# Autodesk Inventor assembly: 胴体_1
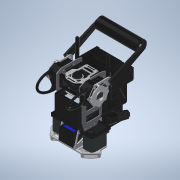
[picture p0: Inventor's stored thumbnail of the model, 180x180]
Saved by Autodesk Inventor 2020 (Build 240168000, 168)
## iProperties
Created: 2016-05-03
Part Number: 胴体_1
Document SubType Name: Assembly
Designer: hiroaki
Mass: 1394.39 g
Surface Area: 4542.63 cm^2
Volume: 847.153 cm^3
Density: 1.64598 g/cm^3
Author: hiroaki
## Documents named in this file (26)
- C:\Users\Masato\Documents\Inventor\CIT Brains_Inventor\OpenPlatform_ver3_0\上半身\胴体\胴体_1.iam
- C:\Users\Masato\Documents\Inventor\CIT Brains_Inventor\OpenPlatform_ver3_0\既製品\B3M11xx.ipt
- C:\Users\Masato\Documents\Inventor\CIT Brains_Inventor\OpenPlatform_ver3_0\既製品\B3M10xx.ipt
- C:\Users\Masato\Documents\Inventor\CIT Brains_Inventor\OpenPlatform_ver3_0\上半身\胴体\胴体_メインフレーム_1_1.ipt
- C:\Users\Masato\Documents\Inventor\CIT Brains_Inventor\OpenPlatform_ver3_0\下半身\付け根ロール\付け根ロール_サブフレーム_1_3.ipt
- C:\Users\Masato\Documents\Inventor\CIT Brains_Inventor\OpenPlatform_ver3_0\上半身\胴体\胴体_メインフレーム_1_2.ipt
- C:\Users\Masato\Documents\Inventor\CIT Brains_Inventor\OpenPlatform_ver3_0\上半身\胴体\胴体_サブフレーム_1_1.ipt
- C:\Users\Masato\Documents\Inventor\CIT Brains_Inventor\OpenPlatform_ver3_0\上半身\胴体\胴体_サブフレーム_1_2.ipt
- C:\Users\Masato\Documents\Inventor\CIT Brains_Inventor\OpenPlatform_ver3_0\上半身\胴体\胴体_サブフレーム_1_3.ipt
- C:\Users\Masato\Documents\Inventor\CIT Brains_Inventor\OpenPlatform_ver3_0\上半身\胴体\胴体_サブフレーム_1_4.ipt
- C:\Users\Masato\Documents\Inventor\CIT Brains_Inventor\OpenPlatform_ver3_0\上半身\胴体\胴体_サブフレーム_1_1_MIR.ipt
- C:\Users\Masato\Documents\Inventor\CIT Brains_Inventor\OpenPlatform_ver3_0\上半身\胴体\胴体_サブフレーム_1_9.ipt
- C:\Users\Masato\Documents\Inventor\CIT Brains_Inventor\OpenPlatform_ver3_0\上半身\胴体\胴体_メインフレーム_1_12.ipt
- C:\Users\Masato\Documents\Inventor\CIT Brains_Inventor\OpenPlatform_ver3_0\上半身\胴体\胴体_メインフレーム_1_13.ipt
- C:\Users\Masato\Documents\Inventor\CIT Brains_Inventor\OpenPlatform_ver3_0\上半身\胴体\胴体_サブフレーム_1_10.ipt
- C:\Users\Masato\Documents\Inventor\CIT Brains_Inventor\OpenPlatform_ver3_0\既製品\MSU-306-03.ipt
- C:\Users\Masato\Documents\Inventor\CIT Brains_Inventor\OpenPlatform_ver3_0\既製品\ALSFB6-66.ipt
- C:\Users\Masato\Documents\Inventor\CIT Brains_Inventor\OpenPlatform_ver3_0\上半身\胴体\胴体_サブフレーム_1_12.ipt
- C:\Users\Masato\Documents\Inventor\CIT Brains_Inventor\OpenPlatform_ver3_0\上半身\胴体\胴体_サブフレーム_1_4_MIR.ipt
- C:\Users\Masato\Documents\Inventor\CIT Brains_Inventor\OpenPlatform_ver3_0\上半身\胴体\RearBumper_Lower.ipt
- C:\Users\Masato\Documents\Inventor\CIT Brains_Inventor\OpenPlatform_ver3_0\上半身\胴体\RearBumper_Lower_MIR.ipt
- C:\Users\Masato\Documents\Inventor\CIT Brains_Inventor\OpenPlatform_ver3_0\上半身\胴体\FrontBumper_MIR.iam
- C:\Users\Masato\Documents\Inventor\CIT Brains_Inventor\OpenPlatform_ver3_0\上半身\胴体\FrontBumper.iam
- C:\Users\Masato\Documents\Inventor\CIT Brains_Inventor\OpenPlatform_ver3_0\既製品\SGB-100.ipt
- C:\Users\Masato\Documents\Inventor\CIT Brains_Inventor\OpenPlatform_ver3_0\上半身\Cockpit\Cockpit.iam
- C:\Users\Masato\Documents\Inventor\CIT Brains_Inventor\OpenPlatform_ver3_0\既製品\AETTF8-130-M3-N3.ipt
## Components (61 placed, 24 different names)
1. 胴体_メインフレーム_1_1:1 — 挿入:1, 挿入:2, 挿入:3, 挿入:4, 挿入:5, 挿入:6, 挿入:43, 挿入:44, 挿入:120, 挿入:121, 挿入:194, 挿入:195, 挿入:196, 挿入:197, 挿入:198, 挿入:199, 挿入:200, 挿入:201, メイト:18
2. 付け根ロール_サブフレーム_1_3:1 — 挿入:218, 挿入:219, 挿入:220, 挿入:221
3. 胴体_メインフレーム_1_2:1 — 挿入:23, 挿入:24, 挿入:25, 挿入:28
4. 胴体_メインフレーム_1_12:1 — 挿入:148, 挿入:149, 挿入:150, 挿入:151, メイト:13, メイト:16
5. 胴体_サブフレーム_1_1:1 — 挿入:43, 挿入:44, メイト:10, メイト:11, 挿入:275, 挿入:276
6. 胴体_サブフレーム_1_2:1 — フラッシュ:1, メイト:3, メイト:4
7. 胴体_サブフレーム_1_3:1 — 挿入:150, 挿入:151, 挿入:162, 挿入:163, 挿入:168, 挿入:169, 挿入:192, 挿入:193, 挿入:228, 挿入:229, メイト:4, 挿入:236, メイト:12, フラッシュ:2
8. 胴体_サブフレーム_1_4:1 — 挿入:57, 挿入:58, 挿入:148, 挿入:149, 挿入:152, 挿入:153, 挿入:206, 挿入:207, 挿入:208, 挿入:209, 挿入:248, 挿入:249, 角度:47, 角度:48
9. 胴体_サブフレーム_1_9:1 — 挿入:133, 挿入:134, 挿入:135
10. 胴体_サブフレーム_1_10:1 — 挿入:173, 挿入:174, 挿入:175, 挿入:176, 挿入:179, 挿入:188, 挿入:189
11. 胴体_サブフレーム_1_12:1 — 挿入:250, 挿入:251
12. 胴体_メインフレーム_1_13:1 — 挿入:188, 挿入:189, 挿入:190, 挿入:191, 挿入:192, 挿入:193, 挿入:277
13. B3M11xx:5 — 挿入:175, 挿入:176, 挿入:179
14. B3M11xx:4 — 挿入:57, 挿入:58, 挿入:133, 挿入:134, 挿入:135, 角度:31, 角度:39
15. B3M11xx:3 — 角度:1, 挿入:130, 挿入:131, 挿入:132, 挿入:264, 挿入:265, 挿入:266
16. B3M11xx:2 — 挿入:2, 挿入:4, 挿入:5, 挿入:23, 挿入:25, 角度:23, 角度:43
17. B3M11xx:1 — 角度:1, 挿入:1, 挿入:3, 挿入:6, 挿入:24, 挿入:28
18. MSU-306-03:1 — 挿入:200, 挿入:218, 角度:27, 角度:29
19. MSU-306-03:2 — 挿入:196, 挿入:222, 角度:25, 角度:28, 角度:43
20. MSU-306-03:3 — 挿入:198, 挿入:220, 角度:29
21. MSU-306-03:4 — 挿入:199, 挿入:219, 角度:30
22. MSU-306-03:5 — 挿入:217, 角度:34, 挿入:272
23. MSU-306-03:6 — 挿入:216, 角度:42, 挿入:271
24. MSU-306-03:7 — 挿入:197, 挿入:225, 角度:26
25. MSU-306-03:8 — 挿入:201, 挿入:221, 角度:28, 角度:30
26. MSU-306-03:9 — 挿入:206, 挿入:212, 角度:40
27. MSU-306-03:10 — 挿入:215, 角度:41, 挿入:269
28. MSU-306-03:11 — 挿入:214, 角度:33, 角度:34, 挿入:270
29. MSU-306-03:12 — 挿入:195, 挿入:224, 角度:25
30. MSU-306-03:13 — 挿入:207, 挿入:213, 角度:32
31. MSU-306-03:14 — 挿入:208, 挿入:211, 角度:31, 角度:32, 角度:33
32. MSU-306-03:15 — 挿入:209, 挿入:210, 角度:39, 角度:40, 角度:41, 角度:42
33. MSU-306-03:16 — 挿入:194, 挿入:223, 角度:23, 角度:26, 角度:27
34. ALSFB6-66:1 — 挿入:229, 挿入:230, メイト:3
35. ALSFB6-66:2 — 挿入:227, 挿入:228, メイト:1, メイト:2
36. ALSFB6-66:3 — メイト:10, メイト:11, 挿入:235, 挿入:236
37. MSU-306-03:17 — 挿入:252, 挿入:262
38. MSU-306-03:18 — 挿入:249, 挿入:251, 角度:48
39. MSU-306-03:19 — 挿入:253, 挿入:263
40. MSU-306-03:20 — 挿入:248, 挿入:250, 角度:47
41. 胴体_サブフレーム_1_12:2 — 挿入:252, 挿入:253, 挿入:279, 挿入:280
42. 胴体_メインフレーム_1_13:2 — 挿入:168, 挿入:169, 挿入:170, 挿入:171, 挿入:173, 挿入:174, 挿入:278
43. 胴体_メインフレーム_1_12:2 — 挿入:152, 挿入:153, 挿入:162, 挿入:163
44. 胴体_メインフレーム_1_12:3 — 挿入:156, 挿入:157, 挿入:267, 挿入:268
45. 胴体_メインフレーム_1_12:4 — 挿入:160, 挿入:161, 挿入:260, 挿入:261, メイト:15, メイト:17
46. 胴体_サブフレーム_1_9:2 — 挿入:130, 挿入:131, 挿入:132
47. 付け根ロール_サブフレーム_1_3:2 — 挿入:222, 挿入:223, 挿入:224, 挿入:225
48. 付け根ロール_サブフレーム_1_3:3 — 挿入:210, 挿入:211, 挿入:212, 挿入:213
49. 付け根ロール_サブフレーム_1_3:4 — 挿入:214, 挿入:215, 挿入:216, 挿入:217
50. 胴体_サブフレーム_1_1_MIR:1 — 挿入:120, 挿入:121, メイト:7, 挿入:273, 挿入:274
51. 胴体_サブフレーム_1_2:2 — メイト:1, フラッシュ:1, メイト:2, メイト:5, メイト:7
52. 胴体_サブフレーム_1_3:2 — 挿入:156, 挿入:157, 挿入:160, 挿入:161, 挿入:170, 挿入:171, 挿入:190, 挿入:191, 挿入:227, 挿入:230, メイト:5, 挿入:235, メイト:14, メイト:19
53. 胴体_サブフレーム_1_4_MIR:1 — 挿入:260, 挿入:261, 挿入:262, 挿入:263, 挿入:264, 挿入:265, 挿入:266, 挿入:267, 挿入:268, 挿入:269, 挿入:270, 挿入:271, 挿入:272
54. RearBumper_Lower:1 — 挿入:275, 挿入:276
55. RearBumper_Lower_MIR:1 — 挿入:273, 挿入:274
56. FrontBumper_MIR:1 [sub-assembly] — メイト:12, メイト:13, メイト:16
57. FrontBumper:1 [sub-assembly] — メイト:14, メイト:15, メイト:17
58. 胴体_サブフレーム_1_10:2 — 挿入:277, 挿入:278
59. SGB-100:1 — 挿入:280
60. Cockpit:1 [sub-assembly] — フラッシュ:2, メイト:18, メイト:19
61. AETTF8-130-M3-N3:1 — 挿入:279
## Relationships (147: Insert 110, Angle 19, Mate 16, Flush 2)
- 角度:1 [Angle] (0 deg): B3M11xx:3 ↔ B3M11xx:1
- 挿入:1 [Insert]: 胴体_メインフレーム_1_1:1 ↔ B3M11xx:1
- 挿入:2 [Insert]: 胴体_メインフレーム_1_1:1 ↔ B3M11xx:2
- 挿入:3 [Insert]: 胴体_メインフレーム_1_1:1 ↔ B3M11xx:1
- 挿入:4 [Insert]: 胴体_メインフレーム_1_1:1 ↔ B3M11xx:2
- 挿入:5 [Insert]: 胴体_メインフレーム_1_1:1 ↔ B3M11xx:2
- 挿入:6 [Insert]: 胴体_メインフレーム_1_1:1 ↔ B3M11xx:1
- 挿入:23 [Insert]: 胴体_メインフレーム_1_2:1 ↔ B3M11xx:2
- 挿入:24 [Insert]: 胴体_メインフレーム_1_2:1 ↔ B3M11xx:1
- 挿入:25 [Insert]: 胴体_メインフレーム_1_2:1 ↔ B3M11xx:2
- 挿入:28 [Insert]: 胴体_メインフレーム_1_2:1 ↔ B3M11xx:1
- 挿入:43 [Insert]: 胴体_メインフレーム_1_1:1 ↔ 胴体_サブフレーム_1_1:1
- 挿入:44 [Insert]: 胴体_メインフレーム_1_1:1 ↔ 胴体_サブフレーム_1_1:1
- 挿入:57 [Insert]: 胴体_サブフレーム_1_4:1 ↔ B3M11xx:4
- 挿入:58 [Insert]: 胴体_サブフレーム_1_4:1 ↔ B3M11xx:4
- 挿入:120 [Insert]: 胴体_メインフレーム_1_1:1 ↔ 胴体_サブフレーム_1_1_MIR:1
- 挿入:121 [Insert]: 胴体_メインフレーム_1_1:1 ↔ 胴体_サブフレーム_1_1_MIR:1
- 挿入:130 [Insert]: B3M11xx:3 ↔ 胴体_サブフレーム_1_9:2
- 挿入:131 [Insert]: B3M11xx:3 ↔ 胴体_サブフレーム_1_9:2
- 挿入:132 [Insert]: B3M11xx:3 ↔ 胴体_サブフレーム_1_9:2
- 挿入:133 [Insert]: 胴体_サブフレーム_1_9:1 ↔ B3M11xx:4
- 挿入:134 [Insert]: 胴体_サブフレーム_1_9:1 ↔ B3M11xx:4
- 挿入:135 [Insert]: 胴体_サブフレーム_1_9:1 ↔ B3M11xx:4
- 挿入:148 [Insert]: 胴体_メインフレーム_1_12:1 ↔ 胴体_サブフレーム_1_4:1
- 挿入:149 [Insert]: 胴体_メインフレーム_1_12:1 ↔ 胴体_サブフレーム_1_4:1
- 挿入:150 [Insert]: 胴体_メインフレーム_1_12:1 ↔ 胴体_サブフレーム_1_3:1
- 挿入:151 [Insert]: 胴体_メインフレーム_1_12:1 ↔ 胴体_サブフレーム_1_3:1
- 挿入:152 [Insert]: 胴体_サブフレーム_1_4:1 ↔ 胴体_メインフレーム_1_12:2
- 挿入:153 [Insert]: 胴体_サブフレーム_1_4:1 ↔ 胴体_メインフレーム_1_12:2
- 挿入:156 [Insert]: 胴体_メインフレーム_1_12:3 ↔ 胴体_サブフレーム_1_3:2
- 挿入:157 [Insert]: 胴体_メインフレーム_1_12:3 ↔ 胴体_サブフレーム_1_3:2
- 挿入:160 [Insert]: 胴体_メインフレーム_1_12:4 ↔ 胴体_サブフレーム_1_3:2
- 挿入:161 [Insert]: 胴体_メインフレーム_1_12:4 ↔ 胴体_サブフレーム_1_3:2
- 挿入:162 [Insert]: 胴体_サブフレーム_1_3:1 ↔ 胴体_メインフレーム_1_12:2
- 挿入:163 [Insert]: 胴体_サブフレーム_1_3:1 ↔ 胴体_メインフレーム_1_12:2
- 挿入:168 [Insert]: 胴体_サブフレーム_1_3:1 ↔ 胴体_メインフレーム_1_13:2
- 挿入:169 [Insert]: 胴体_サブフレーム_1_3:1 ↔ 胴体_メインフレーム_1_13:2
- 挿入:170 [Insert]: 胴体_メインフレーム_1_13:2 ↔ 胴体_サブフレーム_1_3:2
- 挿入:171 [Insert]: 胴体_メインフレーム_1_13:2 ↔ 胴体_サブフレーム_1_3:2
- 挿入:173 [Insert]: 胴体_サブフレーム_1_10:1 ↔ 胴体_メインフレーム_1_13:2
- 挿入:174 [Insert]: 胴体_サブフレーム_1_10:1 ↔ 胴体_メインフレーム_1_13:2
- 挿入:175 [Insert]: 胴体_サブフレーム_1_10:1 ↔ B3M11xx:5
- 挿入:176 [Insert]: 胴体_サブフレーム_1_10:1 ↔ B3M11xx:5
- 挿入:179 [Insert]: 胴体_サブフレーム_1_10:1 ↔ B3M11xx:5
- 挿入:188 [Insert]: 胴体_サブフレーム_1_10:1 ↔ 胴体_メインフレーム_1_13:1
- 挿入:189 [Insert]: 胴体_サブフレーム_1_10:1 ↔ 胴体_メインフレーム_1_13:1
- 挿入:190 [Insert]: 胴体_メインフレーム_1_13:1 ↔ 胴体_サブフレーム_1_3:2
- 挿入:191 [Insert]: 胴体_メインフレーム_1_13:1 ↔ 胴体_サブフレーム_1_3:2
- 挿入:192 [Insert]: 胴体_サブフレーム_1_3:1 ↔ 胴体_メインフレーム_1_13:1
- 挿入:193 [Insert]: 胴体_サブフレーム_1_3:1 ↔ 胴体_メインフレーム_1_13:1
- 挿入:194 [Insert]: 胴体_メインフレーム_1_1:1 ↔ MSU-306-03:16
- 挿入:195 [Insert]: 胴体_メインフレーム_1_1:1 ↔ MSU-306-03:12
- 挿入:196 [Insert]: 胴体_メインフレーム_1_1:1 ↔ MSU-306-03:2
- 挿入:197 [Insert]: 胴体_メインフレーム_1_1:1 ↔ MSU-306-03:7
- 挿入:198 [Insert]: 胴体_メインフレーム_1_1:1 ↔ MSU-306-03:3
- 挿入:199 [Insert]: 胴体_メインフレーム_1_1:1 ↔ MSU-306-03:4
- 挿入:200 [Insert]: 胴体_メインフレーム_1_1:1 ↔ MSU-306-03:1
- 挿入:201 [Insert]: 胴体_メインフレーム_1_1:1 ↔ MSU-306-03:8
- 挿入:206 [Insert]: 胴体_サブフレーム_1_4:1 ↔ MSU-306-03:9
- 挿入:207 [Insert]: 胴体_サブフレーム_1_4:1 ↔ MSU-306-03:13
- 挿入:208 [Insert]: 胴体_サブフレーム_1_4:1 ↔ MSU-306-03:14
- 挿入:209 [Insert]: 胴体_サブフレーム_1_4:1 ↔ MSU-306-03:15
- 挿入:210 [Insert]: MSU-306-03:15 ↔ 付け根ロール_サブフレーム_1_3:3
- 挿入:211 [Insert]: MSU-306-03:14 ↔ 付け根ロール_サブフレーム_1_3:3
- 挿入:212 [Insert]: MSU-306-03:9 ↔ 付け根ロール_サブフレーム_1_3:3
- 挿入:213 [Insert]: MSU-306-03:13 ↔ 付け根ロール_サブフレーム_1_3:3
- 挿入:214 [Insert]: MSU-306-03:11 ↔ 付け根ロール_サブフレーム_1_3:4
- 挿入:215 [Insert]: MSU-306-03:10 ↔ 付け根ロール_サブフレーム_1_3:4
- 挿入:216 [Insert]: MSU-306-03:6 ↔ 付け根ロール_サブフレーム_1_3:4
- 挿入:217 [Insert]: MSU-306-03:5 ↔ 付け根ロール_サブフレーム_1_3:4
- 挿入:218 [Insert]: 付け根ロール_サブフレーム_1_3:1 ↔ MSU-306-03:1
- 挿入:219 [Insert]: 付け根ロール_サブフレーム_1_3:1 ↔ MSU-306-03:4
- 挿入:220 [Insert]: 付け根ロール_サブフレーム_1_3:1 ↔ MSU-306-03:3
- 挿入:221 [Insert]: 付け根ロール_サブフレーム_1_3:1 ↔ MSU-306-03:8
- 挿入:222 [Insert]: MSU-306-03:2 ↔ 付け根ロール_サブフレーム_1_3:2
- 挿入:223 [Insert]: MSU-306-03:16 ↔ 付け根ロール_サブフレーム_1_3:2
- 挿入:224 [Insert]: MSU-306-03:12 ↔ 付け根ロール_サブフレーム_1_3:2
- 挿入:225 [Insert]: MSU-306-03:7 ↔ 付け根ロール_サブフレーム_1_3:2
- 角度:23 [Angle] (0 deg): B3M11xx:2 ↔ MSU-306-03:16
- 角度:25 [Angle] (0 deg): MSU-306-03:2 ↔ MSU-306-03:12
- 角度:26 [Angle] (0 deg): MSU-306-03:7 ↔ MSU-306-03:16
- 角度:27 [Angle] (0 deg): MSU-306-03:1 ↔ MSU-306-03:16
- 角度:28 [Angle] (0 deg): MSU-306-03:2 ↔ MSU-306-03:8
- 角度:29 [Angle] (0 deg): MSU-306-03:1 ↔ MSU-306-03:3
- 角度:30 [Angle] (0 deg): MSU-306-03:4 ↔ MSU-306-03:8
- 角度:31 [Angle] (0 deg): B3M11xx:4 ↔ MSU-306-03:14
- 角度:32 [Angle] (0 deg): MSU-306-03:13 ↔ MSU-306-03:14
- 角度:33 [Angle] (0 deg): MSU-306-03:11 ↔ MSU-306-03:14
- 角度:34 [Angle] (0 deg): MSU-306-03:5 ↔ MSU-306-03:11
- 挿入:227 [Insert]: ALSFB6-66:2 ↔ 胴体_サブフレーム_1_3:2
- 挿入:228 [Insert]: 胴体_サブフレーム_1_3:1 ↔ ALSFB6-66:2
- 挿入:229 [Insert]: 胴体_サブフレーム_1_3:1 ↔ ALSFB6-66:1
- 挿入:230 [Insert]: ALSFB6-66:1 ↔ 胴体_サブフレーム_1_3:2
- メイト:1 [Mate] (0.005 mm): ALSFB6-66:2 ↔ 胴体_サブフレーム_1_2:2
- フラッシュ:1 [Flush]: 胴体_サブフレーム_1_2:1 ↔ 胴体_サブフレーム_1_2:2
- メイト:2 [Mate] (0.05 mm): ALSFB6-66:2 ↔ 胴体_サブフレーム_1_2:2
- メイト:3 [Mate] (0.005 mm): 胴体_サブフレーム_1_2:1 ↔ ALSFB6-66:1
- メイト:4 [Mate]: 胴体_サブフレーム_1_2:1 ↔ 胴体_サブフレーム_1_3:1
- メイト:5 [Mate]: 胴体_サブフレーム_1_2:2 ↔ 胴体_サブフレーム_1_3:2
- メイト:7 [Mate]: 胴体_サブフレーム_1_1_MIR:1 ↔ 胴体_サブフレーム_1_2:2
- メイト:10 [Mate] (0.005 mm): 胴体_サブフレーム_1_1:1 ↔ ALSFB6-66:3
- メイト:11 [Mate] (0.005 mm): 胴体_サブフレーム_1_1:1 ↔ ALSFB6-66:3
- 挿入:235 [Insert]: ALSFB6-66:3 ↔ 胴体_サブフレーム_1_3:2
- 挿入:236 [Insert]: 胴体_サブフレーム_1_3:1 ↔ ALSFB6-66:3
- 挿入:248 [Insert]: 胴体_サブフレーム_1_4:1 ↔ MSU-306-03:20
- 挿入:249 [Insert]: 胴体_サブフレーム_1_4:1 ↔ MSU-306-03:18
- 挿入:250 [Insert]: 胴体_サブフレーム_1_12:1 ↔ MSU-306-03:20
- 挿入:251 [Insert]: 胴体_サブフレーム_1_12:1 ↔ MSU-306-03:18
- 挿入:252 [Insert]: MSU-306-03:17 ↔ 胴体_サブフレーム_1_12:2
- 挿入:253 [Insert]: MSU-306-03:19 ↔ 胴体_サブフレーム_1_12:2
- 角度:39 [Angle] (0 deg): B3M11xx:4 ↔ MSU-306-03:15
- 角度:40 [Angle] (0 deg): MSU-306-03:9 ↔ MSU-306-03:15
- 角度:41 [Angle] (0 deg): MSU-306-03:10 ↔ MSU-306-03:15
- 角度:42 [Angle] (0 deg): MSU-306-03:6 ↔ MSU-306-03:15
- 角度:43 [Angle] (0 deg): B3M11xx:2 ↔ MSU-306-03:2
- 角度:47 [Angle] (0 deg): 胴体_サブフレーム_1_4:1 ↔ MSU-306-03:20
- 角度:48 [Angle] (0 deg): 胴体_サブフレーム_1_4:1 ↔ MSU-306-03:18
- 挿入:260 [Insert]: 胴体_メインフレーム_1_12:4 ↔ 胴体_サブフレーム_1_4_MIR:1
- 挿入:261 [Insert]: 胴体_メインフレーム_1_12:4 ↔ 胴体_サブフレーム_1_4_MIR:1
- 挿入:262 [Insert]: MSU-306-03:17 ↔ 胴体_サブフレーム_1_4_MIR:1
- 挿入:263 [Insert]: MSU-306-03:19 ↔ 胴体_サブフレーム_1_4_MIR:1
- 挿入:264 [Insert]: B3M11xx:3 ↔ 胴体_サブフレーム_1_4_MIR:1
- 挿入:265 [Insert]: B3M11xx:3 ↔ 胴体_サブフレーム_1_4_MIR:1
- 挿入:266 [Insert]: B3M11xx:3 ↔ 胴体_サブフレーム_1_4_MIR:1
- 挿入:267 [Insert]: 胴体_メインフレーム_1_12:3 ↔ 胴体_サブフレーム_1_4_MIR:1
- 挿入:268 [Insert]: 胴体_メインフレーム_1_12:3 ↔ 胴体_サブフレーム_1_4_MIR:1
- 挿入:269 [Insert]: MSU-306-03:10 ↔ 胴体_サブフレーム_1_4_MIR:1
- 挿入:270 [Insert]: MSU-306-03:11 ↔ 胴体_サブフレーム_1_4_MIR:1
- 挿入:271 [Insert]: MSU-306-03:6 ↔ 胴体_サブフレーム_1_4_MIR:1
- 挿入:272 [Insert]: MSU-306-03:5 ↔ 胴体_サブフレーム_1_4_MIR:1
- メイト:12 [Mate]: 胴体_サブフレーム_1_3:1 ↔ FrontBumper_MIR:1
- メイト:13 [Mate]: 胴体_メインフレーム_1_12:1 ↔ FrontBumper_MIR:1
- メイト:14 [Mate]: 胴体_サブフレーム_1_3:2 ↔ FrontBumper:1
- メイト:15 [Mate]: 胴体_メインフレーム_1_12:4 ↔ FrontBumper:1
- 挿入:273 [Insert]: 胴体_サブフレーム_1_1_MIR:1 ↔ RearBumper_Lower_MIR:1
- 挿入:274 [Insert]: 胴体_サブフレーム_1_1_MIR:1 ↔ RearBumper_Lower_MIR:1
- 挿入:275 [Insert]: 胴体_サブフレーム_1_1:1 ↔ RearBumper_Lower:1
- 挿入:276 [Insert]: 胴体_サブフレーム_1_1:1 ↔ RearBumper_Lower:1
- メイト:16 [Mate]: 胴体_メインフレーム_1_12:1 ↔ FrontBumper_MIR:1
- メイト:17 [Mate]: 胴体_メインフレーム_1_12:4 ↔ FrontBumper:1
- 挿入:277 [Insert]: 胴体_メインフレーム_1_13:1 ↔ 胴体_サブフレーム_1_10:2
- 挿入:278 [Insert]: 胴体_メインフレーム_1_13:2 ↔ 胴体_サブフレーム_1_10:2
- フラッシュ:2 [Flush] (-12.5 mm): 胴体_サブフレーム_1_3:1 ↔ Cockpit:1
- メイト:18 [Mate]: 胴体_メインフレーム_1_1:1 ↔ Cockpit:1
- メイト:19 [Mate]: 胴体_サブフレーム_1_3:2 ↔ Cockpit:1
- 挿入:279 [Insert]: 胴体_サブフレーム_1_12:2 ↔ AETTF8-130-M3-N3:1
- 挿入:280 [Insert] (2.5 mm): 胴体_サブフレーム_1_12:2 ↔ SGB-100:1
